# Autodesk Inventor assembly: Water Drainage for Red Pump
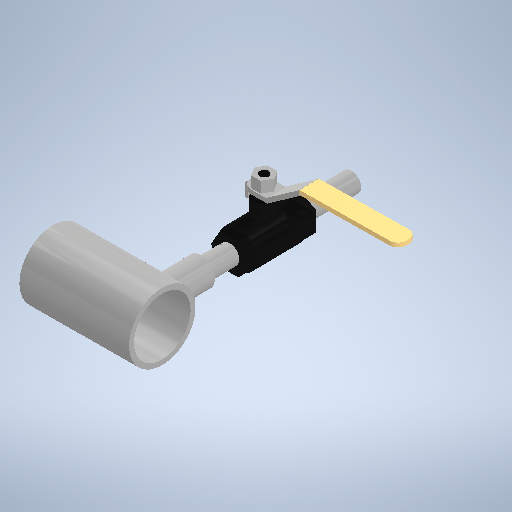
[picture p0: Inventor's stored thumbnail of the model, 512x512]
Saved by Autodesk Inventor 2027 (Build 310192000, 192)
## iProperties
Created: 2026-08-31
Part Number: Water Drainage for Red Pump
Document SubType Name: Assembly
Designer: IG2
Author: IG2
## Documents named in this file (4)
- C:\Users\ig2\Desktop\Inventor stuff on your own\Water Drainage for Red Pump.iam
- C:\Users\ig2\Desktop\Inventor stuff on your own\red pump valve water pipe v4.ipt
- C:\Users\ig2\Desktop\Inventor stuff on your own\red pump valve lever v2.ipt
- C:\Users\ig2\Desktop\Inventor stuff on your own\red pump pipe connector for water valve v4.ipt
## Components (3 placed, 3 different names)
1. red pump valve water pipe v4:1 — Rotational:1, Rigid:1
2. red pump valve lever v2:1 — Rotational:1
3. red pump pipe connector for water valve v4:1 — Rigid:1
## Relationships (2: RevoluteJoint 1, WeldJoint 1)
- Rotational:1 [RevoluteJoint] (88.9 mm): red pump valve water pipe v4:1 ↔ red pump valve lever v2:1
- Rigid:1 [WeldJoint] (-25.4 mm): red pump valve water pipe v4:1 ↔ red pump pipe connector for water valve v4:1
